# Autodesk Inventor assembly: gear180_03
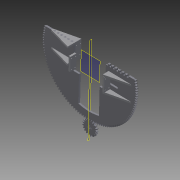
[picture p0: Inventor's stored thumbnail of the model, 180x180]
Saved by Autodesk Inventor 2013 (Build 170138000, 138)
## iProperties
Created: 2013-02-22
Part Number: gear180_03
Document SubType Name: Assembly
Designer: Nano
Author: Nano
## Documents named in this file (10)
- C:\Users\Nano\Documents\InventorByron\InventorMasterProject\gyroPhone01\gear180_03.iam
- C:\Users\Nano\Documents\InventorByron\InventorMasterProject\gyroPhone01\gear180_03\Design Accelerator\Spur Gears1.iam
- C:\Users\Nano\Documents\InventorByron\InventorMasterProject\gyroPhone01\brace01.ipt
- C:\Users\Nano\Documents\InventorByron\InventorMasterProject\gyroPhone01\brace02.ipt
- C:\Users\Nano\Documents\InventorByron\InventorMasterProject\gyroPhone01\basePlate01.ipt
- C:\Users\Nano\Documents\InventorByron\InventorMasterProject\gyroPhone01\brace01_MIR.ipt
- C:\Users\Nano\Documents\InventorByron\InventorMasterProject\gyroPhone01\brace02_MIR.ipt
- C:\Users\Nano\Documents\InventorByron\InventorMasterProject\gyroPhone01\basePlate01_MIR.ipt
- C:\Users\Nano\Documents\InventorByron\InventorMasterProject\gyroPhone01\basePlate01_MIR1.ipt
- C:\Users\Nano\Documents\InventorByron\InventorMasterProject\gyroPhone01\basePlate01_MIR_MIR.ipt
## Components (9 placed, 9 different names)
1. Spur Gears:1 [sub-assembly] — Flush:1, Flush:1, Mate:1, Flush:2, Mate:2, Mate:3, Flush:3, Mate:4, Flush:4, Mate:6, Angle:1
2. brace01:1 — Flush:1, Flush:1, Mate:1
3. brace02:1 — Flush:2, Mate:2, Mate:5, Flush:4
4. basePlate01:1 — Mate:3, Flush:3, Mate:4, Mate:5
5. brace01_MIR:1
6. brace02_MIR:1
7. basePlate01_MIR:1
8. basePlate01_MIR1:1
9. basePlate01_MIR_MIR:1
## Relationships (12: Mate 6, Flush 5, Angle 1)
- Flush:1: Spur Gears:1 ↔ brace01:1
- Flush:1: Spur Gears:1 ↔ brace01:1
- Mate:1: Spur Gears:1 ↔ brace01:1
- Flush:2: Spur Gears:1 ↔ brace02:1
- Mate:2: Spur Gears:1 ↔ brace02:1
- Mate:3: Spur Gears:1 ↔ basePlate01:1
- Flush:3: Spur Gears:1 ↔ basePlate01:1
- Mate:4: Spur Gears:1 ↔ basePlate01:1
- Mate:5: brace02:1 ↔ basePlate01:1
- Flush:4: Spur Gears:1 ↔ brace02:1
- Mate:6: Spur Gears:1
- Angle:1 (0 deg): Spur Gears:1
